# Autodesk Inventor assembly: tarot680pro_vib_damp
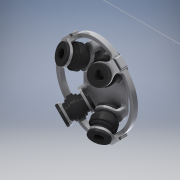
[picture p0: Inventor's stored thumbnail of the model, 180x180]
Saved by Autodesk Inventor 2017 SP1 (Build 210196100, 196)
## iProperties
Created: 2016-07-15
Part Number: tarot680pro_vib_damp
Document SubType Name: Assembly
Designer: Mert
Mass: 21.7148 g
Surface Area: 269.322 cm^2
Volume: 20.6573 cm^3
Density: 1.05119 g/cm^3
Author: Mert
## Documents named in this file (5)
- C:\Users\Mert\AppData\Local\Autodesk\Autodesk Sync\Cloud\mert.ozata@kozagold.com\tarot680pro_vib_damp\tarot680pro_vib_damp.iam
- C:\Users\Mert\AppData\Local\Autodesk\Autodesk Sync\Cloud\mert.ozata@kozagold.com\tarot680pro_vib_damp\tarot_PCB_center.ipt
- C:\Users\Mert\AppData\Local\Autodesk\Autodesk Sync\Cloud\mert.ozata@kozagold.com\tarot680pro_vib_damp\bottom_frame.ipt
- C:\Users\Mert\AppData\Local\Autodesk\Autodesk Sync\Cloud\mert.ozata@kozagold.com\tarot680pro_vib_damp\top_frame.ipt
- C:\Users\Mert\AppData\Local\Autodesk\Autodesk Sync\Cloud\mert.ozata@kozagold.com\tarot680pro_vib_damp\lastik.ipt
## Components (7 placed, 4 different names)
1. tarot_PCB_center:1
2. bottom_frame:1 — Mate:2, Mate:3, Mate:4, Mate:5, Mate:6, Mate:7, Mate:8, Mate:9
3. top_frame:1 — Mate:1, Mate:10
4. lastik:1 — Mate:1, Mate:2, Mate:9
5. lastik:2 — Mate:3, Mate:4
6. lastik:3 — Mate:7, Mate:8
7. lastik:4 — Mate:5, Mate:6, Mate:10
## Relationships (10: Mate 10)
- Mate:1: top_frame:1 ↔ lastik:1
- Mate:2: bottom_frame:1 ↔ lastik:1
- Mate:3: bottom_frame:1 ↔ lastik:2
- Mate:4: bottom_frame:1 ↔ lastik:2
- Mate:5: bottom_frame:1 ↔ lastik:4
- Mate:6: bottom_frame:1 ↔ lastik:4
- Mate:7: bottom_frame:1 ↔ lastik:3
- Mate:8: bottom_frame:1 ↔ lastik:3
- Mate:9: bottom_frame:1 ↔ lastik:1
- Mate:10: top_frame:1 ↔ lastik:4
## Named parameters: offset = 0.5 mm
